# Autodesk Inventor assembly: RoomWallAssembly
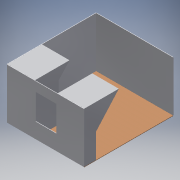
[picture p0: Inventor's stored thumbnail of the model, 180x180]
Saved by Autodesk Inventor 2018 (Build 220112000, 112)
## iProperties
Created: 2019-04-28
Part Number: RoomWallAssembly
Document SubType Name: Assembly
Designer: snipe
Author: snipe
## Documents named in this file (10)
- C:\Users\snipe\Documents\FrileyResidenceHallRoomCAD\4517\RoomWallAssembly.iam
- C:\Users\snipe\Documents\FrileyResidenceHallRoomCAD\4517\Footprint.ipt
- C:\Users\snipe\Documents\FrileyResidenceHallRoomCAD\4517\NorthWall.ipt
- C:\Users\snipe\Documents\FrileyResidenceHallRoomCAD\4517\SouthWall.ipt
- C:\Users\snipe\Documents\FrileyResidenceHallRoomCAD\4517\EastWall.ipt
- C:\Users\snipe\Documents\FrileyResidenceHallRoomCAD\4517\WestWall.ipt
- C:\Users\snipe\Documents\FrileyResidenceHallRoomCAD\4517\SouthWestWallBlock.ipt
- C:\Users\snipe\Documents\FrileyResidenceHallRoomCAD\4517\SouthWestWallBlockAngle.ipt
- C:\Users\snipe\Documents\FrileyResidenceHallRoomCAD\4517\SouthEastWallBlock.ipt
- C:\Users\snipe\Documents\FrileyResidenceHallRoomCAD\4517\SouthEastWallBlockAngle.ipt
## Components (9 placed, 9 different names)
1. Footprint:1 — Mate:1, Flush:1, Mate:4, Mate:3, Flush:2, Mate:5, Mate:6, Flush:3, Mate:7, Mate:8, Flush:4, Mate:9, Mate:12, Mate:18
2. NorthWall:1 — Mate:4, Mate:3, Flush:2
3. SouthWall:1 — Mate:1, Flush:1, Mate:7, Mate:10, Mate:13, Mate:16, Mate:19
4. EastWall:1 — Mate:5, Mate:6, Flush:3, Mate:17, Mate:20
5. WestWall:1 — Mate:8, Flush:4, Mate:9, Mate:11, Mate:14
6. SouthWestWallBlock:1 — Mate:10, Mate:11, Mate:12, Mate:15
7. SouthWestWallBlockAngle:1 — Mate:13, Mate:14, Mate:15
8. SouthEastWallBlock:1 — Mate:16, Mate:17, Mate:18, Mate:21
9. SouthEastWallBlockAngle:1 — Mate:19, Mate:20, Mate:21
## Relationships (24: Mate 20, Flush 4)
- Mate:1: Footprint:1 ↔ SouthWall:1
- Flush:1: Footprint:1 ↔ SouthWall:1
- Mate:4: Footprint:1 ↔ NorthWall:1
- Mate:3: Footprint:1 ↔ NorthWall:1
- Flush:2: Footprint:1 ↔ NorthWall:1
- Mate:5: Footprint:1 ↔ EastWall:1
- Mate:6: Footprint:1 ↔ EastWall:1
- Flush:3: Footprint:1 ↔ EastWall:1
- Mate:7: Footprint:1 ↔ SouthWall:1
- Mate:8: Footprint:1 ↔ WestWall:1
- Flush:4: Footprint:1 ↔ WestWall:1
- Mate:9: Footprint:1 ↔ WestWall:1
- Mate:10: SouthWall:1 ↔ SouthWestWallBlock:1
- Mate:11: WestWall:1 ↔ SouthWestWallBlock:1
- Mate:12: Footprint:1 ↔ SouthWestWallBlock:1
- Mate:13: SouthWall:1 ↔ SouthWestWallBlockAngle:1
- Mate:14: WestWall:1 ↔ SouthWestWallBlockAngle:1
- Mate:15: SouthWestWallBlock:1 ↔ SouthWestWallBlockAngle:1
- Mate:16: SouthWall:1 ↔ SouthEastWallBlock:1
- Mate:17: EastWall:1 ↔ SouthEastWallBlock:1
- Mate:18: Footprint:1 ↔ SouthEastWallBlock:1
- Mate:19: SouthWall:1 ↔ SouthEastWallBlockAngle:1
- Mate:20: EastWall:1 ↔ SouthEastWallBlockAngle:1
- Mate:21: SouthEastWallBlock:1 ↔ SouthEastWallBlockAngle:1
